# Autodesk Inventor assembly: Assembly5
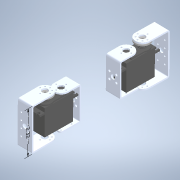
[picture p0: Inventor's stored thumbnail of the model, 180x180]
Saved by Autodesk Inventor 2022 (Build 260153000, 153)
## iProperties
Created: 2022-04-22
Part Number: Assembly5
Document SubType Name: Assembly
Designer: HP
Author: HP
## Documents named in this file (9)
- C:\Users\HP\Documents\Inventor\spider\Assembly5.iam
- C:\Users\HP\Downloads\tower-pro-mg996r-servo-1.snapshot.3\Tower Pro MG996R.ipt
- C:\Users\HP\Downloads\Servo horn v2.ipt
- C:\Users\HP\Downloads\demir1.ipt
- C:\Users\HP\Downloads\demir2.ipt
- C:\Users\HP\Downloads\tower-pro-mg996r-servo-1.snapshot.3\Tower Pro MG996R_CPY1.ipt
- C:\Users\HP\Downloads\Servo horn v2_CPY1.ipt
- C:\Users\HP\Downloads\demir1_CPY1.ipt
- C:\Users\HP\Downloads\demir2_CPY1.ipt
## Components (8 placed, 8 different names)
1. Tower Pro MG996R:1 — Mate:1, Flush:2, Mate:4, Mate:5, Mate:6
2. Servo horn v2:1 — Mate:5, Mate:6
3. demir1:1 — Flush:6
4. demir2:1 — Mate:1, Flush:2, Mate:4, Flush:4, Flush:5
5. Tower Pro MG996R_CPY1:1 — Mate:7, Mate:8, Mate:9, Flush:3, Mate:10
6. Servo horn v2_CPY1:1 — Mate:7, Mate:8
7. demir1_CPY1:1 — Flush:6
8. demir2_CPY1:1 — Mate:9, Flush:3, Mate:10, Flush:4, Flush:5
## Relationships (13: Mate 8, Flush 5)
- Mate:1: Tower Pro MG996R:1 ↔ demir2:1
- Flush:2: Tower Pro MG996R:1 ↔ demir2:1
- Mate:4 (2.413 mm): Tower Pro MG996R:1 ↔ demir2:1
- Mate:5 (6.604 mm): Tower Pro MG996R:1 ↔ Servo horn v2:1
- Mate:6: Tower Pro MG996R:1 ↔ Servo horn v2:1
- Mate:7: Tower Pro MG996R_CPY1:1 ↔ Servo horn v2_CPY1:1
- Mate:8 (6.604 mm): Tower Pro MG996R_CPY1:1 ↔ Servo horn v2_CPY1:1
- Mate:9 (2.413 mm): Tower Pro MG996R_CPY1:1 ↔ demir2_CPY1:1
- Flush:3: Tower Pro MG996R_CPY1:1 ↔ demir2_CPY1:1
- Mate:10: Tower Pro MG996R_CPY1:1 ↔ demir2_CPY1:1
- Flush:4: demir2:1 ↔ demir2_CPY1:1
- Flush:5: demir2:1 ↔ demir2_CPY1:1
- Flush:6: demir1:1 ↔ demir1_CPY1:1
